# Autodesk Inventor assembly: my trunk assembly
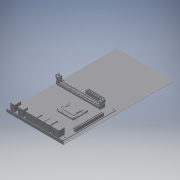
[picture p0: Inventor's stored thumbnail of the model, 180x180]
Saved by Autodesk Inventor 2018 (Build 220112000, 112)
## iProperties
Created: 2018-06-19
Part Number: my trunk assembly
Document SubType Name: Assembly
Designer: John Viljoen
Author: John Viljoen
## Documents named in this file (3)
- C:\Users\John Viljoen\Documents\Inventor\computer project\my trunk assembly.iam
- C:\Users\John Viljoen\Documents\Inventor\computer project\my trunk.ipt
- C:\Users\John Viljoen\Documents\Inventor\computer project\Mini-ITX Mobo.ipt
## Components (2 placed, 2 different names)
1. my trunk:1 — Mate:1, Mate:2, Angle:1
2. Mini-ITX Mobo:1 — Mate:1, Mate:2, Angle:1
## Relationships (3: Mate 2, Angle 1)
- Mate:1 (10 mm): my trunk:1 ↔ Mini-ITX Mobo:1
- Mate:2: my trunk:1 ↔ Mini-ITX Mobo:1
- Angle:1 (0 deg): my trunk:1 ↔ Mini-ITX Mobo:1
